# Autodesk Inventor assembly: Left Hook Whole Assembly_v2
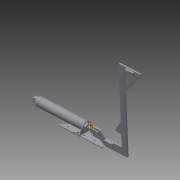
[picture p0: Inventor's stored thumbnail of the model, 180x180]
Saved by Autodesk Inventor 2013 (Build 170138000, 138)
## iProperties
Created: 2013-03-16
Part Number: Left Hook Whole Assembly_v2
Document SubType Name: Assembly
Designer: Arpan
Author: Arpan
## Documents named in this file (4)
- C:\Users\Arpan\Documents\GitHub\frc2013CAD\Midwest Climber\Left Hook Whole Assembly_v2.iam
- C:\Users\Arpan\Documents\GitHub\frc2013CAD\Midwest Climber\Left Hook Encoder Assembly.iam
- C:\Users\Arpan\Documents\GitHub\frc2013CAD\Midwest Climber\Piston Bracket Assembly.iam
- C:\Users\Arpan\Documents\GitHub\frc2013CAD\Midwest Climber\Ninja cylinder support bracket.ipt
## Components (3 placed, 3 different names)
1. Left Hook Encoder Assembly:1 [sub-assembly] — Mate:7, Mate:8, Mate:9
2. Piston Bracket Assembly:1 [sub-assembly] — Mate:4, Mate:5, Mate:6, Mate:7, Mate:8, Mate:9
3. Ninja cylinder support bracket:1 — Mate:4, Mate:5, Mate:6
## Relationships (6: Mate 6)
- Mate:4: Piston Bracket Assembly:1 ↔ Ninja cylinder support bracket:1
- Mate:5: Piston Bracket Assembly:1 ↔ Ninja cylinder support bracket:1
- Mate:6: Piston Bracket Assembly:1 ↔ Ninja cylinder support bracket:1
- Mate:7: Left Hook Encoder Assembly:1 ↔ Piston Bracket Assembly:1
- Mate:8: Left Hook Encoder Assembly:1 ↔ Piston Bracket Assembly:1
- Mate:9: Left Hook Encoder Assembly:1 ↔ Piston Bracket Assembly:1
